# Autodesk Inventor assembly: SCTW12
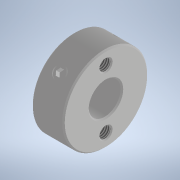
[picture p0: Inventor's stored thumbnail of the model, 180x180]
Saved by Autodesk Inventor 2021 (Build 250183000, 183)
## iProperties
Category: PARTsolutions
Company: MISUMI
Created: 2025-04-29
Part Number: SCTW12
Catalog Web Link: www.cadenas.de
Description: SCTW, PSCTW, SSCTW-Shaft Collars - Set Screw, with 2 Holes
Vendor: MISUMI
Document SubType Name: Assembly
Designer: psAdmin
Manufacturer: MISUMI
Mass: 7.81903 g
Surface Area: 36.5329 cm^2
Volume: 7.81903 cm^3
Density: 1 g/cm^3
Title: SCTW12
Author: Cadenas PARTsolutions
Comments: Shaft Collars - Set Screw, with 2 Holes
PSOL_IDENT_0: {$CADENAS_DATA/23d-libs/misumi/metric/03_set_collars/sctw_asmtab.prj},184 {VTYP=3D},{STYP=ASSTAB},{N
PSOL_IDENT_1: B=SCTW12},{LINA=SCTW12},{NN=SCTW, PSCTW, SSCTW},{DATE=02.06.2021 03:00:04},{GEOMDATE=25.12.2015 07:4
PSOL_IDENT_2: 9:56},{VERSION=},{LINEID=70},{WBVAR=MAT,ST},{WBNUMERIC=}  {NB=SCTW12},{LINA=SCTW12},{KT=DUMMY},{PN=S
PSOL_IDENT_3: CTW12},{TYPE=SCTW},{MAT=1045},{ST=Black Oxide},{AC=Set Screws 2 Pcs.},{D=12},{B=12},{D1=32},{P=22},{
PSOL_IDENT_4: M=M5x5},{THMD=5},{THDMIN=4.134},{M1=M5},{C=0.5},{ST0='Black Oxide','Black Oxide','Electroless Nickel
PSOL_IDENT_5: Plating','Electroless Nickel Plating'},{L=5},{PPATH=sctw/sctw_asmtpl.prj}
NB: SCTW12
NN: SCTW, PSCTW, SSCTW
NT: Shaft Collars - Set Screw, with 2 Holes
NBSYN: $PN.
LINA: SCTW12
CATALOG: Misumi
PN: SCTW12
MAT: S45C Equivalent
ST: Black Oxide
AC: Set Screws 2 Pcs.
D: 12
B: 12
D1: 32
P: 22
M: M5x5
M1: M5
SUPPLIER: MISUMI
ARTICLENO: SCTW12
BOMINFO: SCTW12
CREATOR: CADENAS GmbH
## Documents named in this file (3)
- e:\temp\worker_COMMON_340\temp\tmp_860_28_Gm8B0\format_0\SCTW12.iam
- e:\temp\worker_COMMON_340\temp\tmp_860_28_Gm8B0\format_0\SCTW12b.ipt
- e:\temp\worker_COMMON_340\temp\tmp_860_28_Gm8B0\format_0\Hexagon socket set screw with flat point DIN 913 - M5x5.ipt
## Components (3 placed, 2 different names)
1. SCTW12b:1 — body_set_v_XY@1 <-> IP1_XY@2, body_set_v_Z@1 <-> IP1_Z@2, body_set_v_YZ@1 <-> IP1_YZ@2, body_set_h_XY@1 <-> IP1_XY@3, body_set_h_Z@1 <-> IP1_Z@3, body_set_h_YZ@1 <-> IP1_YZ@3
2. Hexagon socket set screw with flat point DIN 913 - M5x5:1 — body_set_v_XY@1 <-> IP1_XY@2, body_set_v_Z@1 <-> IP1_Z@2, body_set_v_YZ@1 <-> IP1_YZ@2
3. Hexagon socket set screw with flat point DIN 913 - M5x5:2 — body_set_h_XY@1 <-> IP1_XY@3, body_set_h_Z@1 <-> IP1_Z@3, body_set_h_YZ@1 <-> IP1_YZ@3
## Relationships (6: Mate 3, Angle 2, Flush 1)
- body_set_v_XY@1 <-> IP1_XY@2 [Mate]: SCTW12b:1 ↔ Hexagon socket set screw with flat point DIN 913 - M5x5:1
- body_set_v_Z@1 <-> IP1_Z@2 [Mate]: SCTW12b:1 ↔ Hexagon socket set screw with flat point DIN 913 - M5x5:1
- body_set_v_YZ@1 <-> IP1_YZ@2 [Angle] (0 deg): SCTW12b:1 ↔ Hexagon socket set screw with flat point DIN 913 - M5x5:1
- body_set_h_XY@1 <-> IP1_XY@3 [Flush]: SCTW12b:1 ↔ Hexagon socket set screw with flat point DIN 913 - M5x5:2
- body_set_h_Z@1 <-> IP1_Z@3 [Mate]: SCTW12b:1 ↔ Hexagon socket set screw with flat point DIN 913 - M5x5:2
- body_set_h_YZ@1 <-> IP1_YZ@3 [Angle] (0 deg): SCTW12b:1 ↔ Hexagon socket set screw with flat point DIN 913 - M5x5:2
